# Autodesk Inventor assembly: Stopa v2 P
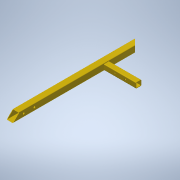
[picture p0: Inventor's stored thumbnail of the model, 180x180]
Saved by Autodesk Inventor 2021 (Build 250183000, 183)
## iProperties
Created: 2024-04-18
Part Number: Stopa v2 P
Document SubType Name: Assembly
Designer: Michal
Author: Michal
## Documents named in this file (3)
- C:\Users\Michal\Documents\GitHub\PNW_PhotoBoothFrame_3D\Stopa v2 P.iam
- C:\Users\Michal\Documents\GitHub\PNW_PhotoBoothFrame_3D\Stopa v2 profil 1.ipt
- C:\Users\Michal\Documents\GitHub\PNW_PhotoBoothFrame_3D\Stopa v2 profil 3.ipt
## Components (2 placed, 2 different names)
1. Stopa v2 profil 3:1 — Mate:11, Mate:12, Mate:14, Mate:15
2. Stopa v2 profil 1:1 — Mate:12, Mate:13, Flush:5, Mate:15
## Relationships (6: Mate 5, Flush 1)
- Mate:11: Stopa v2 profil 3:1
- Mate:12: Stopa v2 profil 3:1 ↔ Stopa v2 profil 1:1
- Mate:13: Stopa v2 profil 1:1
- Flush:5: Stopa v2 profil 1:1
- Mate:14: Stopa v2 profil 3:1
- Mate:15 (150 mm): Stopa v2 profil 3:1 ↔ Stopa v2 profil 1:1
